# Autodesk Inventor assembly: Montiert
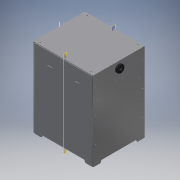
[picture p0: Inventor's stored thumbnail of the model, 180x180]
Saved by Autodesk Inventor 2018 (Build 220112000, 112)
## iProperties
Created: 2017-11-12
Part Number: Montiert
Material: Generisch
Document SubType Name: Assembly
## Documents named in this file (9)
- C:\git\RoKu-ProjectX01\Konstruktion\Montiert.iam
- C:\git\RoKu-ProjectX01\Konstruktion\Brenner.ipt
- C:\git\RoKu-ProjectX01\Konstruktion\Gegenhalter.ipt
- C:\git\RoKu-ProjectX01\Konstruktion\BrennerBrennTeil.ipt
- C:\git\RoKu-ProjectX01\Konstruktion\Back.ipt
- C:\git\RoKu-ProjectX01\Konstruktion\Seite.ipt
- C:\git\RoKu-ProjectX01\Konstruktion\Front.ipt
- C:\git\RoKu-ProjectX01\Konstruktion\Deckel.ipt
- C:\git\RoKu-ProjectX01\Konstruktion\MutterMitUScheibe.ipt
## Components (20 placed, 8 different names)
1. Brenner:1 — Fluchtend:1, Fluchtend:2, Fluchtend:3, Passend:1, Passend:2, Fluchtend:4, Passend:3, Passend:4
2. Gegenhalter:1 — Passend:1, Passend:2
3. BrennerBrennTeil:1 — Fluchtend:4
4. Back:1 — Passend:3, Passend:4, Passend:5, Passend:6, Fluchtend:6, Fluchtend:7, Passend:7, Fluchtend:8, Fluchtend:9, Passend:15, Passend:16, Passend:17, Passend:18, Passend:19, Passend:20, Passend:21, Passend:22
5. Seite:1 — Passend:6, Fluchtend:6, Fluchtend:7, Passend:8, Fluchtend:11, Passend:9, Fluchtend:12, Passend:11, Passend:12, Passend:13, Passend:14
6. Seite:2 — Passend:7, Fluchtend:8, Fluchtend:9, Fluchtend:10, Passend:23, Passend:24, Passend:25, Passend:26
7. Front:1 — Passend:8, Fluchtend:10, Fluchtend:11, Passend:10, Passend:27, Passend:28, Passend:29, Passend:30, Passend:31, Passend:32, Passend:33, Passend:34
8. Deckel:1 — Passend:9, Fluchtend:12, Passend:10
9. MutterMitUScheibe:1 — Passend:19, Passend:20
10. MutterMitUScheibe:2 — Passend:21, Passend:22
11. MutterMitUScheibe:3 — Passend:23, Passend:24
12. MutterMitUScheibe:4 — Passend:25, Passend:26
13. MutterMitUScheibe:5 — Passend:29, Passend:30
14. MutterMitUScheibe:6 — Passend:33, Passend:34
15. MutterMitUScheibe:7 — Passend:31, Passend:32
16. MutterMitUScheibe:8 — Passend:27, Passend:28
17. MutterMitUScheibe:9 — Passend:17, Passend:18
18. MutterMitUScheibe:10 — Passend:11, Passend:12
19. MutterMitUScheibe:11 — Passend:13, Passend:14
20. MutterMitUScheibe:12 — Passend:15, Passend:16
## Relationships (45: Mate 34, Flush 11)
- Fluchtend:1 [Flush]: Brenner:1
- Fluchtend:2 [Flush]: Brenner:1
- Fluchtend:3 [Flush]: Brenner:1
- Passend:1 [Mate] (2 mm): Brenner:1 ↔ Gegenhalter:1
- Passend:2 [Mate]: Brenner:1 ↔ Gegenhalter:1
- Fluchtend:4 [Flush]: Brenner:1 ↔ BrennerBrennTeil:1
- Passend:3 [Mate]: Brenner:1 ↔ Back:1
- Passend:4 [Mate] (-10 mm): Brenner:1 ↔ Back:1
- Passend:5 [Mate]: Back:1
- Passend:6 [Mate]: Back:1 ↔ Seite:1
- Fluchtend:6 [Flush]: Back:1 ↔ Seite:1
- Fluchtend:7 [Flush]: Back:1 ↔ Seite:1
- Passend:7 [Mate]: Back:1 ↔ Seite:2
- Fluchtend:8 [Flush]: Back:1 ↔ Seite:2
- Fluchtend:9 [Flush]: Back:1 ↔ Seite:2
- Passend:8 [Mate]: Seite:1 ↔ Front:1
- Fluchtend:10 [Flush]: Seite:2 ↔ Front:1
- Fluchtend:11 [Flush]: Seite:1 ↔ Front:1
- Passend:9 [Mate]: Seite:1 ↔ Deckel:1
- Fluchtend:12 [Flush]: Seite:1 ↔ Deckel:1
- Passend:10 [Mate]: Front:1 ↔ Deckel:1
- Passend:11 [Mate]: Seite:1 ↔ MutterMitUScheibe:10
- Passend:12 [Mate]: Seite:1 ↔ MutterMitUScheibe:10
- Passend:13 [Mate]: Seite:1 ↔ MutterMitUScheibe:11
- Passend:14 [Mate]: Seite:1 ↔ MutterMitUScheibe:11
- Passend:15 [Mate]: Back:1 ↔ MutterMitUScheibe:12
- Passend:16 [Mate]: Back:1 ↔ MutterMitUScheibe:12
- Passend:17 [Mate]: Back:1 ↔ MutterMitUScheibe:9
- Passend:18 [Mate]: Back:1 ↔ MutterMitUScheibe:9
- Passend:19 [Mate]: Back:1 ↔ MutterMitUScheibe:1
- Passend:20 [Mate]: Back:1 ↔ MutterMitUScheibe:1
- Passend:21 [Mate]: Back:1 ↔ MutterMitUScheibe:2
- Passend:22 [Mate]: Back:1 ↔ MutterMitUScheibe:2
- Passend:23 [Mate]: Seite:2 ↔ MutterMitUScheibe:3
- Passend:24 [Mate]: Seite:2 ↔ MutterMitUScheibe:3
- Passend:25 [Mate]: Seite:2 ↔ MutterMitUScheibe:4
- Passend:26 [Mate]: Seite:2 ↔ MutterMitUScheibe:4
- Passend:27 [Mate]: Front:1 ↔ MutterMitUScheibe:8
- Passend:28 [Mate]: Front:1 ↔ MutterMitUScheibe:8
- Passend:29 [Mate]: Front:1 ↔ MutterMitUScheibe:5
- Passend:30 [Mate]: Front:1 ↔ MutterMitUScheibe:5
- Passend:31 [Mate]: Front:1 ↔ MutterMitUScheibe:7
- Passend:32 [Mate]: Front:1 ↔ MutterMitUScheibe:7
- Passend:33 [Mate]: Front:1 ↔ MutterMitUScheibe:6
- Passend:34 [Mate]: Front:1 ↔ MutterMitUScheibe:6
